# Autodesk Inventor assembly: L clamp
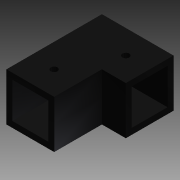
[picture p0: Inventor's stored thumbnail of the model, 180x180]
Saved by Autodesk Inventor 2015 (Build 190159000, 159)
## iProperties
Created: 2013-11-23
Part Number: L clamp
Document SubType Name: Assembly
Designer: Jesse Stevenson
Author: Jesse Stevenson
## Documents named in this file (3)
- C:\Users\jesse\Desktop\robot\L clamp.iam
- C:\Users\jesse\Desktop\robot\L clamp - bottom.ipt
- C:\Users\jesse\Desktop\robot\L clamp - top.ipt
## Components (2 placed, 2 different names)
1. L clamp - bottom:1 — Mate:1, Flush:1, Flush:2
2. L clamp - top:1 — Mate:1, Flush:1, Flush:2
## Relationships (3: Flush 2, Mate 1)
- Mate:1: L clamp - bottom:1 ↔ L clamp - top:1
- Flush:1: L clamp - bottom:1 ↔ L clamp - top:1
- Flush:2: L clamp - bottom:1 ↔ L clamp - top:1
